# Autodesk Inventor assembly: test_dzialania
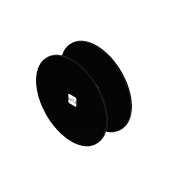
[picture p0: Inventor's stored thumbnail of the model, 180x180]
Saved by Autodesk Inventor 2017 (Build 210142000, 142)
## iProperties
Created: 2018-02-23
Part Number: test_dzialania
Document SubType Name: Assembly
Designer: Dazzyl
Author: Dazzyl
## Documents named in this file (9)
- C:\Users\Dazzyl\Desktop\test_dzialania.iam
- C:\Users\Dazzyl\Desktop\plate_beta.ipt
- C:\Users\Dazzyl\Desktop\spreyna_beta.ipt
- C:\Users\Dazzyl\Desktop\test_dzialania\AIP\FEA\cfhemf334.fins
- C:\Users\Dazzyl\Desktop\test_dzialania\AIP\FEA\cfhemf334.fsat
- C:\Users\Dazzyl\Desktop\test_dzialania\AIP\FEA\cfhemf334.ftes
- C:\Users\Dazzyl\Desktop\test_dzialania\AIP\FEA\cfhemf334.fwiz
- C:\Users\Dazzyl\Desktop\test_dzialania\AIP\FEA\cfhemf340.fmsh
- C:\Users\Dazzyl\Desktop\test_dzialania\AIP\FEA\cfhemf341.fres
## Components (3 placed, 2 different names)
1. plate_beta:1 — Mate:1, Mate:3, Mate:4
2. spreyna_beta:1 — Mate:1, Mate:2
3. plate_beta:2 — Mate:2, Mate:3, Mate:4
## Relationships (4: Mate 4)
- Mate:1: plate_beta:1 ↔ spreyna_beta:1
- Mate:2: spreyna_beta:1 ↔ plate_beta:2
- Mate:3: plate_beta:1 ↔ plate_beta:2
- Mate:4 (50 mm): plate_beta:1 ↔ plate_beta:2
## Named parameters: sa_0 = 0, sa_1 = -0.01, sa_2 = 0
note: some values were not read from the file. Shown as the stored number, unit unknown: "sa_0", "sa_1", "sa_2".
